# Autodesk Inventor assembly: main
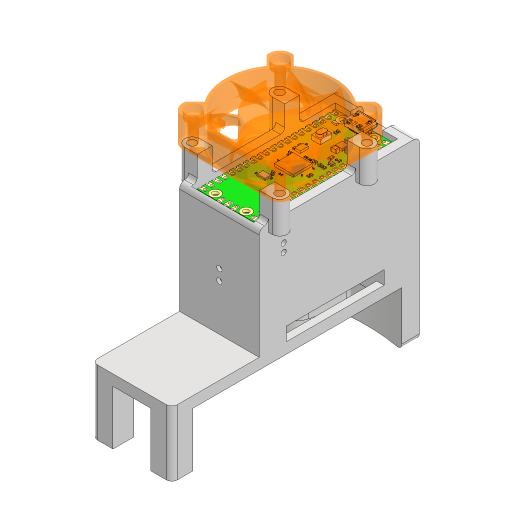
[picture p0: Inventor's stored thumbnail of the model, 512x512]
Saved by Autodesk Inventor 2024.3 (Build 283343000, 343)
## iProperties
Created: 2023-02-06
Part Number: main
Document SubType Name: Assembly
Designer: taka2
Author: taka2
## Documents named in this file (7)
- C:\Users\taka\OneDrive\ドキュメント\04Myproject\Modeling\Inventor\smart_rimocon\main.iam
- C:\Users\taka\OneDrive\ドキュメント\04Myproject\Modeling\Inventor\smart_rimocon\base.ipt
- C:\Users\taka\OneDrive\ドキュメント\04Myproject\Modeling\Inventor\smart_rimocon\stick.ipt
- C:\Users\taka\OneDrive\ドキュメント\04Myproject\Modeling\Inventor\template\サーボモータ.ipt
- C:\Users\taka\OneDrive\ドキュメント\04Myproject\Modeling\Inventor\template\サーボホーン.ipt
- C:\Users\taka\OneDrive\ドキュメント\04Myproject\Modeling\Inventor\smart_rimocon\raspberrypipico\Raspberry Pi Pico-R3\Raspberry Pi Pico-R3\Raspberry Pi Pico-R3.iam
- C:\Users\taka\OneDrive\ドキュメント\04Myproject\Modeling\Inventor\smart_rimocon\fun\CPU - -KF0410-01\CPU - -KF0410-01\CPU - -KF0410-01.iam
## Components (6 placed, 6 different names)
1. base:1 — リジッド:3, リジッド:5, リジッド:6
2. サーボモータ:1 — リジッド:3, 回転:1
3. サーボホーン:1 — リジッド:4, 回転:1
4. stick:1 — リジッド:4
5. Raspberry Pi Pico-R3:1 [sub-assembly] — リジッド:5
6. CPU - -KF0410-01:1 [sub-assembly] — リジッド:6
## Relationships (5: WeldJoint 4, RevoluteJoint 1)
- リジッド:3 [WeldJoint]: base:1 ↔ サーボモータ:1
- リジッド:4 [WeldJoint]: サーボホーン:1 ↔ stick:1
- 回転:1 [RevoluteJoint] (2.5 mm): サーボモータ:1 ↔ サーボホーン:1
- リジッド:5 [WeldJoint]: base:1 ↔ Raspberry Pi Pico-R3:1
- リジッド:6 [WeldJoint]: base:1 ↔ CPU - -KF0410-01:1
